# Autodesk Inventor assembly: openmv4_h7_base_® ã¬®«ç ­¨î
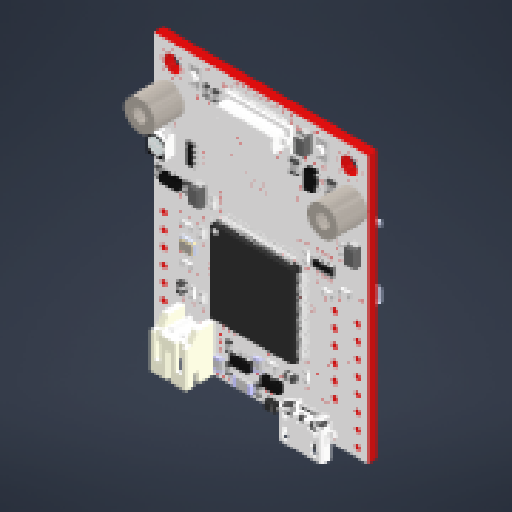
[picture p0: Inventor's stored thumbnail of the model, 512x512]
Saved by Autodesk Inventor 2023.2 (Build 272271030, 271C)
## iProperties
Created: 2023-01-17
Part Number: openmv4_h7_base_® ã¬®«ç ­¨î
Document SubType Name: Assembly
Designer: Elias Braun
Author: Elias Braun
Revision Number: ANY
## Documents named in this file (23)
- C:\Users\Elias Braun\Nextcloud2\RoboCup2023\Cam\OpenMV H7\OpenMVH7openmv4_h7_base.iam
- C:\Users\Elias Braun\Nextcloud2\RoboCup2023\Cam\OpenMV H7\OpenMVH7base.ipt
- C:\Users\Elias Braun\Nextcloud2\RoboCup2023\Cam\OpenMV H7\OpenMVH7C0603K_C0603K_0603.ipt
- C:\Users\Elias Braun\Nextcloud2\RoboCup2023\Cam\OpenMV H7\OpenMVH70805.ipt
- C:\Users\Elias Braun\Nextcloud2\RoboCup2023\Cam\OpenMV H7\OpenMVH7C0805K_C0805K.ipt
- C:\Users\Elias Braun\Nextcloud2\RoboCup2023\Cam\OpenMV H7\OpenMVH7cap3216h160.ipt
- C:\Users\Elias Braun\Nextcloud2\RoboCup2023\Cam\OpenMV H7\OpenMVH7SOD323_BAT54HT1G.ipt
- C:\Users\Elias Braun\Nextcloud2\RoboCup2023\Cam\OpenMV H7\OpenMVH7Capacitor 0603.ipt
- C:\Users\Elias Braun\Nextcloud2\RoboCup2023\Cam\OpenMV H7\OpenMVH71206.ipt
- C:\Users\Elias Braun\Nextcloud2\RoboCup2023\Cam\OpenMV H7\OpenMVH7LED SMD RGB.ipt
- C:\Users\Elias Braun\Nextcloud2\RoboCup2023\Cam\OpenMV H7\OpenMVH7LED 1206 IR.ipt
- C:\Users\Elias Braun\Nextcloud2\RoboCup2023\Cam\OpenMV H7\OpenMVH7SOT 23.ipt
- C:\Users\Elias Braun\Nextcloud2\RoboCup2023\Cam\OpenMV H7\OpenMVH7Resistor 0603.ipt
- C:\Users\Elias Braun\Nextcloud2\RoboCup2023\Cam\OpenMV H7\OpenMVH7R0603_SJR.ipt
- C:\Users\Elias Braun\Nextcloud2\RoboCup2023\Cam\OpenMV H7\OpenMVH7EXBV8V.ipt
- C:\Users\Elias Braun\Nextcloud2\RoboCup2023\Cam\OpenMV H7\OpenMVH7User Library-LQFP100-3.iam
- C:\Users\Elias Braun\Nextcloud2\RoboCup2023\Cam\OpenMV H7\OpenMVH7SOT 23-5.ipt
- C:\Users\Elias Braun\Nextcloud2\RoboCup2023\Cam\OpenMV H7\OpenMVH7UJ2-MIBH2-4-SMT_Defaut.iam
- C:\Users\Elias Braun\Nextcloud2\RoboCup2023\Cam\OpenMV H7\OpenMVH71040310811_USD1040310811.ipt
- C:\Users\Elias Braun\Nextcloud2\RoboCup2023\Cam\OpenMV H7\OpenMVH7DF12-36DS-0.5V.ipt
- C:\Users\Elias Braun\Nextcloud2\RoboCup2023\Cam\OpenMV H7\OpenMVH7S2B-PH-K-S(LF)(SN).ipt
- C:\Users\Elias Braun\Nextcloud2\RoboCup2023\Cam\OpenMV H7\OpenMVH7Crystal-SM2520-4.ipt
- C:\Users\Elias Braun\Nextcloud2\RoboCup2023\Cam\OpenMV H7\OpenMVH7Standoff metal 5x2.5mm_.ipt
## Components (50 placed, 50 different names)
1. base_® ã¬®«ç ­¨î_14 — Mate:1, Mate:2, Mate:3, Mate:4
2. C0603K_C0603K_0603_15
3. C0603K_C0603K_0603_16
4. 0805_17
5. 0805_18
6. C0805K_C0805K_19
7. C0805K_C0805K_20
8. C0603K_C0603K_0603_21
9. C0603K_C0603K_0603_22
10. C0603K_C0603K_0603_23
11. C0603K_C0603K_0603_24
12. C0603K_C0603K_0603_25
13. C0603K_C0603K_0603_26
14. C0603K_C0603K_0603_27
15. cap3216h160_28
16. cap3216h160_29
17. cap3216h160_30
18. C0603K_C0603K_0603_31
19. C0603K_C0603K_0603_32
20. C0603K_C0603K_0603_33
21. C0603K_C0603K_0603_34
22. SOD323_BAT54HT1G_35
23. Capacitor 0603_39
24. Capacitor 0603_40
25. 1206_41
26. LED SMD RGB_42
27. LED 1206 IR_43
28. LED 1206 IR_44
29. SOT 23_45
30. SOT 23_46
31. Resistor 0603_47
32. Resistor 0603_48
33. Resistor 0603_49
34. Resistor 0603_50
35. Resistor 0603_51
36. R0603_SJR_52
37. R0603_SJR_53
38. EXBV8V_54
39. EXBV8V_55
40. EXBV8V_56
41. User Library-LQFP100-3_57 [sub-assembly]
42. SOT 23-5_58
43. SOT 23-5_59
44. UJ2-MIBH2-4-SMT_Defaut_60 [sub-assembly]
45. 1040310811_USD1040310811_® ã¬®«ç ­¨î_61
46. DF12-36DS-0.5V_® ã¬®«ç ­¨î_62
47. S2B-PH-K-S(LF)(SN)_® ã¬®«ç ­¨î_63
48. Crystal-SM2520-4_64
49. Standoff metal 5x2.5mm_® ã¬®«ç ­¨î_65 — Mate:3, Mate:4
50. Standoff metal 5x2.5mm_® ã¬®«ç ­¨î_66 — Mate:1, Mate:2
## Relationships (4: Mate 4)
- Mate:1: base_® ã¬®«ç ­¨î_14 ↔ Standoff metal 5x2.5mm_® ã¬®«ç ­¨î_66
- Mate:2: base_® ã¬®«ç ­¨î_14 ↔ Standoff metal 5x2.5mm_® ã¬®«ç ­¨î_66
- Mate:3: base_® ã¬®«ç ­¨î_14 ↔ Standoff metal 5x2.5mm_® ã¬®«ç ­¨î_65
- Mate:4: base_® ã¬®«ç ­¨î_14 ↔ Standoff metal 5x2.5mm_® ã¬®«ç ­¨î_65
